# Autodesk Inventor assembly: HM1_FIXT2-002_CAM1
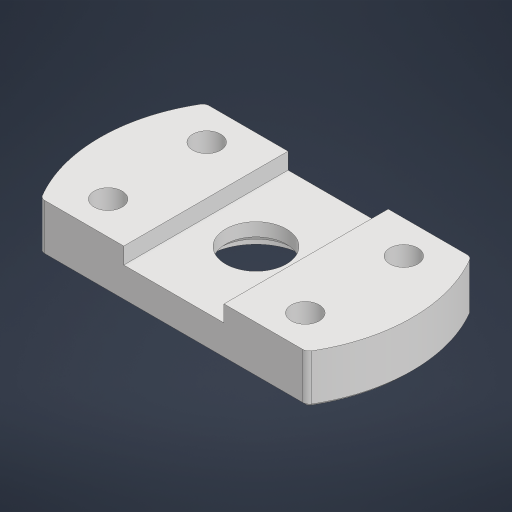
[picture p0: Inventor's stored thumbnail of the model, 512x512]
Saved by Autodesk Inventor 2024.3 (Build 283343000, 343)
## iProperties
Created: 2024-10-21
Part Number: HM1_FIXT2-002_CAM1
Document SubType Name: Assembly
Designer: fablabadmin
Author: fablabadmin
## Documents named in this file (7)
- C:\Users\fablabadmin\Documents\_Benjamin_S\_3dCAD\HHVerkstad\Hammer1\_FIXT2\_002_CAM1\HM1_FIXT2-002_CAM1.iam
- C:\Users\fablabadmin\Documents\_Benjamin_S\_3dCAD\_Config\KemmlerVise\OP1-KemmlerVise.iam
- C:\Users\fablabadmin\Documents\_Benjamin_S\_3dCAD\_Config\KemmlerVise\OP2-KemmlerVise.iam
- C:\Users\fablabadmin\Documents\Inventor\Content Center Files\R2024\en-US\StandardJaw\JawSTD-Aluminum 6061.ipt
- C:\Users\fablabadmin\Documents\_Benjamin_S\_3dCAD\HHVerkstad\Hammer1\_FIXT2\HM1_FIXT2-002.ipt
- C:\Users\fablabadmin\Documents\_Benjamin_S\_3dCAD\HHVerkstad\Hammer1\_FIXT2\_002_CAM1\SquareStock.ipt
- C:\Users\fablabadmin\Documents\_Benjamin_S\_3dCAD\_Config\_CAM_SIM\FixtureParts\parallels3mm.xlsx
## Components (8 placed, 5 different names)
1. HM1_FIXT2-002:1 — Flush:7, Mate:10, Mate:11, Mate:12, Mate:14
2. SquareStock:1 — Flush:5, Flush:6, Flush:7, Mate:7, Mate:8, Mate:9
3. OP1-KemmlerVise:1 [sub-assembly] — Mate:4, Mate:5, Flush:3, Mate:6, Mate:9, Flush:8
4. JawStandard JawSTD-Aluminum 6061:1 — Mate:4, Flush:3, Flush:4, Mate:6, Mate:7
5. JawStandard JawSTD-Aluminum 6061:2 — Mate:5, Flush:4, Mate:8
6. OP2-KemmlerVise:1 [sub-assembly] — Mate:1, Mate:2, Flush:1, Mate:3, Mate:12, Mate:13, Mate:15
7. JawStandard JawSTD-Aluminum 6061:3 — Mate:1, Flush:1, Flush:2, Mate:3, Mate:10
8. JawStandard JawSTD-Aluminum 6061:4 — Mate:2, Flush:2, Mate:11
## Relationships (24: Mate 16, Flush 8)
- Mate:1: OP2-KemmlerVise:1 ↔ JawStandard JawSTD-Aluminum 6061:3
- Mate:2: OP2-KemmlerVise:1 ↔ JawStandard JawSTD-Aluminum 6061:4
- Flush:1: OP2-KemmlerVise:1 ↔ JawStandard JawSTD-Aluminum 6061:3
- Flush:2: JawStandard JawSTD-Aluminum 6061:3 ↔ JawStandard JawSTD-Aluminum 6061:4
- Mate:3: OP2-KemmlerVise:1 ↔ JawStandard JawSTD-Aluminum 6061:3
- Mate:4: OP1-KemmlerVise:1 ↔ JawStandard JawSTD-Aluminum 6061:1
- Mate:5: OP1-KemmlerVise:1 ↔ JawStandard JawSTD-Aluminum 6061:2
- Flush:3: OP1-KemmlerVise:1 ↔ JawStandard JawSTD-Aluminum 6061:1
- Flush:4: JawStandard JawSTD-Aluminum 6061:1 ↔ JawStandard JawSTD-Aluminum 6061:2
- Mate:6: OP1-KemmlerVise:1 ↔ JawStandard JawSTD-Aluminum 6061:1
- Flush:5: SquareStock:1
- Flush:6: SquareStock:1
- Flush:7 (-1 mm): HM1_FIXT2-002:1 ↔ SquareStock:1
- Mate:7: SquareStock:1 ↔ JawStandard JawSTD-Aluminum 6061:1
- Mate:8: SquareStock:1 ↔ JawStandard JawSTD-Aluminum 6061:2
- Mate:9 (38 mm): SquareStock:1 ↔ OP1-KemmlerVise:1
- Flush:8: OP1-KemmlerVise:1
- Mate:10: HM1_FIXT2-002:1 ↔ JawStandard JawSTD-Aluminum 6061:3
- Mate:11: HM1_FIXT2-002:1 ↔ JawStandard JawSTD-Aluminum 6061:4
- Mate:12 (38 mm): HM1_FIXT2-002:1 ↔ OP2-KemmlerVise:1
- Mate:13: OP2-KemmlerVise:1
- Mate:14: HM1_FIXT2-002:1
- Mate:15: OP2-KemmlerVise:1
- Mate:16
## Named parameters: PRL13 = 13 mm, PRL16 = 16 mm, PRL19 = 19 mm, PRL22 = 22 mm, PRL28 = 28 mm, PRL31 = 31 mm, PRL35 = 35 mm, PRL38 = 38 mm, PRL41 = 41 mm
